# Autodesk Inventor assembly: 감속기어2
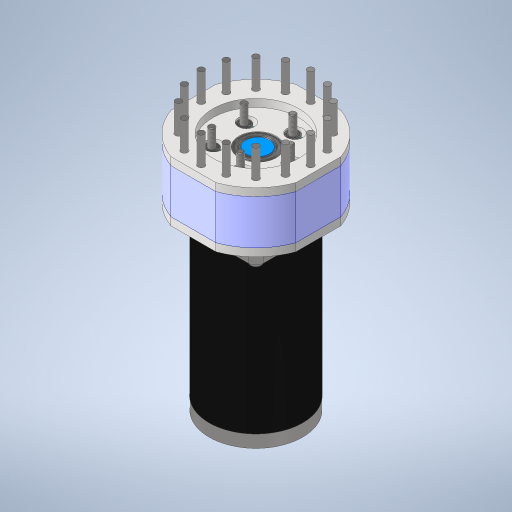
[picture p0: Inventor's stored thumbnail of the model, 512x512]
Saved by Autodesk Inventor 2023 (Build 270158000, 158)
## iProperties
Created: 2022-06-21
Part Number: 감속기어2
Document SubType Name: Assembly
Designer: user
Author: user
## Documents named in this file (3)
- C:\Users\user\Desktop\Baymax-main\설계\출력 부품\감속기어2.iam
- C:\Users\user\Desktop\Baymax-main\설계\출력 부품\감속기어1.iam
- C:\Users\user\Desktop\Baymax-main\설계\출력 부품\감속기어1 - 하우징 상단 커버.ipt
## Components (2 placed, 2 different names)
1. 감속기어1:1 [sub-assembly] — 메이트:1
2. 감속기어1 - 하우징 상단 커버:1 — 메이트:1
## Relationships (1: Mate 1)
- 메이트:1 [Mate]: 감속기어1:1 ↔ 감속기어1 - 하우징 상단 커버:1
